# Autodesk Inventor assembly: Montagem1
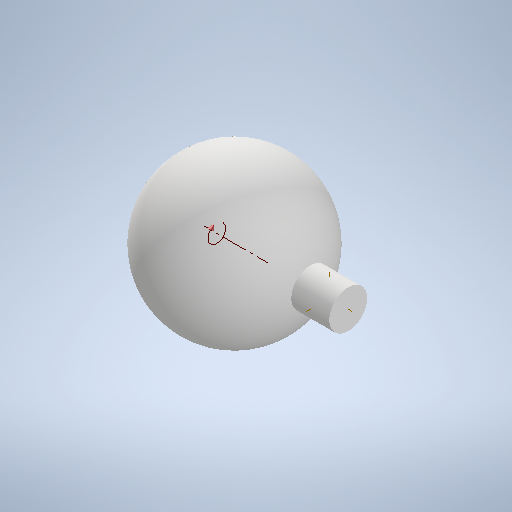
[picture p0: Inventor's stored thumbnail of the model, 512x512]
Saved by Autodesk Inventor 2026 (Build 300175000, 175)
## iProperties
Created: 2025-03-25
Part Number: Montagem1
Document SubType Name: Assembly
Designer: Carlos Dias
Author: Carlos Dias
## Documents named in this file (3)
- C:\Users\Carlos Dias\Documents\Formação-TEARCI\UFCDs\5134 - Robótica _ Fundamentos\Material De Apoio\Assembly\Montagem1.iam
- C:\Users\Carlos Dias\Documents\Formação-TEARCI\UFCDs\5134 - Robótica _ Fundamentos\Material De Apoio\Assembly\peca_011_001.ipt
- C:\Users\Carlos Dias\Documents\Formação-TEARCI\UFCDs\5134 - Robótica _ Fundamentos\Material De Apoio\Assembly\peca_008_001.ipt
## Components (2 placed, 2 different names)
1. peca_011_001:1 — Mate:1, Mate:2, Flush:1, Tangent:1
2. peca_008_001:1 — Mate:3, Tangent:1
## Relationships (5: Mate 3, Flush 1, Tangent 1)
- Mate:1: peca_011_001:1
- Mate:2: peca_011_001:1
- Flush:1: peca_011_001:1
- Mate:3: peca_008_001:1
- Tangent:1: peca_011_001:1 ↔ peca_008_001:1
